# Autodesk Inventor assembly: Z Belt Drive Shaft
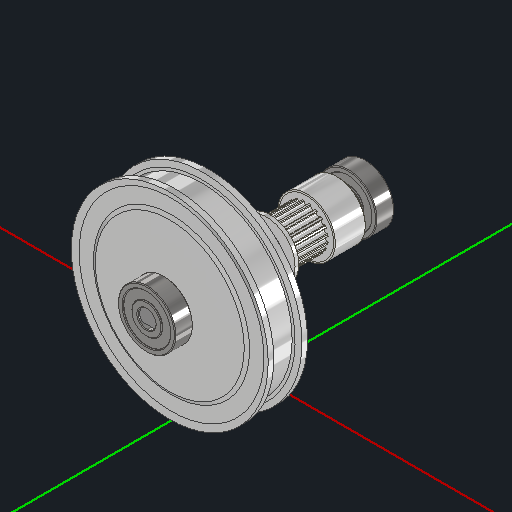
[picture p0: Inventor's stored thumbnail of the model, 512x512]
Saved by Autodesk Inventor 2022 (Build 260153000, 153)
## iProperties
Created: 2022-03-12
Part Number: Z Belt Drive Shaft
Document SubType Name: Assembly
Designer: sleib
Author: sleib
## Documents named in this file (6)
- C:\Users\sleib\Projekte\Voron-2\CAD\Inventor\Z-Belt Drive-Shaft.iam
- C:\Users\sleib\Projekte\Voron-2\CAD\Inventor\Original\5x50 Shaft - With Flat.ipt
- C:\Users\sleib\Projekte\Voron-2\CAD\Inventor\Bearing 625-2RS.ipt
- C:\Users\sleib\Projekte\Voron-2\CAD\Inventor\M5 Spacer (1mm).ipt
- C:\Users\sleib\Projekte\Voron-2\CAD\Inventor\GT2 80T Pulley (6mm).ipt
- C:\Users\sleib\Projekte\Voron-2\CAD\Inventor\GT2 20T Pulley (9mm).ipt
## Components (10 placed, 5 different names)
1. 5x50 Shaft - With Flat:1 — Passend:1, Passend:2, Passend:3, Fluchtend:1, Fluchtend:2, Passend:4, Passend:5, Passend:6, Passend:7, Passend:12, Passend:13
2. Bearing 625-2RS:1 — Passend:3, Fluchtend:1, Passend:16
3. Bearing 625-2RS:2 — Passend:2, Passend:10, Passend:11
4. Bearing 625-2RS:3 — Passend:1, Fluchtend:2
5. M5 Spacer (1mm):1 — Passend:4, Passend:9, Passend:14
6. M5 Spacer (1mm):2 — Passend:5, Passend:9, Passend:10
7. M5 Spacer (1mm):3 — Passend:6, Passend:8, Passend:11
8. M5 Spacer (1mm):4 — Passend:7, Passend:8, Passend:15
9. GT2 80T Pulley (6mm):1 — Passend:13, Passend:14, Passend:16
10. GT2 20T Pulley (9mm):1 — Passend:12, Passend:15
## Relationships (18: Mate 16, Flush 2)
- Passend:1 [Mate]: 5x50 Shaft - With Flat:1 ↔ Bearing 625-2RS:3
- Passend:2 [Mate]: 5x50 Shaft - With Flat:1 ↔ Bearing 625-2RS:2
- Passend:3 [Mate]: 5x50 Shaft - With Flat:1 ↔ Bearing 625-2RS:1
- Fluchtend:1 [Flush] (-0.6 mm): 5x50 Shaft - With Flat:1 ↔ Bearing 625-2RS:1
- Fluchtend:2 [Flush] (-0.6 mm): 5x50 Shaft - With Flat:1 ↔ Bearing 625-2RS:3
- Passend:4 [Mate]: 5x50 Shaft - With Flat:1 ↔ M5 Spacer (1mm):1
- Passend:5 [Mate]: 5x50 Shaft - With Flat:1 ↔ M5 Spacer (1mm):2
- Passend:6 [Mate]: 5x50 Shaft - With Flat:1 ↔ M5 Spacer (1mm):3
- Passend:7 [Mate]: 5x50 Shaft - With Flat:1 ↔ M5 Spacer (1mm):4
- Passend:8 [Mate]: M5 Spacer (1mm):3 ↔ M5 Spacer (1mm):4
- Passend:9 [Mate]: M5 Spacer (1mm):1 ↔ M5 Spacer (1mm):2
- Passend:10 [Mate]: Bearing 625-2RS:2 ↔ M5 Spacer (1mm):2
- Passend:11 [Mate]: Bearing 625-2RS:2 ↔ M5 Spacer (1mm):3
- Passend:12 [Mate]: 5x50 Shaft - With Flat:1 ↔ GT2 20T Pulley (9mm):1
- Passend:13 [Mate]: 5x50 Shaft - With Flat:1 ↔ GT2 80T Pulley (6mm):1
- Passend:14 [Mate]: M5 Spacer (1mm):1 ↔ GT2 80T Pulley (6mm):1
- Passend:15 [Mate]: M5 Spacer (1mm):4 ↔ GT2 20T Pulley (9mm):1
- Passend:16 [Mate] (1.5 mm): Bearing 625-2RS:1 ↔ GT2 80T Pulley (6mm):1
